# Autodesk Inventor assembly: rapoukAssemblyv2
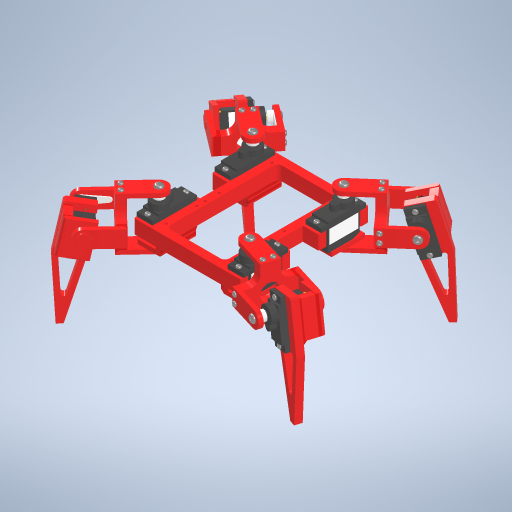
[picture p0: Inventor's stored thumbnail of the model, 512x512]
Saved by Autodesk Inventor 2024 (Build 280153000, 153)
## iProperties
Created: 2024-02-06
Part Number: rapoukAssemblyv2
Document SubType Name: Weldment
Designer: Roman Suk
Weld Material: Welded Aluminum-6061
Author: Roman Suk
## Documents named in this file (9)
- C:\Users\Roman Suk\Documents\Ročníkovka SŠ\CD\Technická dokumentace\rapoukAssemblyv2.iam
- C:\Users\Roman Suk\Documents\Ročníkovka SŠ\CD\Technická dokumentace\rapoukBaseAssemblyv1.iam
- C:\Users\Roman Suk\Documents\Ročníkovka SŠ\CD\Technická dokumentace\сервопривод EMAX ES08MA.ipt
- C:\Users\Roman Suk\Documents\Ročníkovka SŠ\CD\Technická dokumentace\rapoukMiddleLegAssemblyv0.iam
- C:\Users\Roman Suk\Documents\Ročníkovka SŠ\CD\Technická dokumentace\rapoukLegAssemblyv0.iam
- C:\Users\Roman Suk\Documents\Ročníkovka SŠ\CD\Technická dokumentace\rapoukServoLegv0.ipt
- C:\Users\Roman Suk\Documents\Ročníkovka SŠ\CD\Technická dokumentace\rapoukMiddleLeg2v3.ipt
- C:\Users\Roman Suk\Documents\Ročníkovka SŠ\CD\Technická dokumentace\rapoukHexagonScrewM2,5v0.ipt
- C:\Users\Roman Suk\Documents\Ročníkovka SŠ\CD\Technická dokumentace\rapoukHexagonScrewM2v0.ipt
## Components (73 placed, 8 different names)
1. rapoukBaseAssemblyv1:1 [sub-assembly] — Rotational:2, Rotational:4, Rotational:6, Rotational:8, Mate:66, Insert:37, Insert:38, Mate:67, Insert:39, Insert:40, Mate:69, Insert:41, Insert:42, Mate:70, Insert:43, Insert:44
2. сервопривод EMAX ES08MA:1 — Mate:69, Insert:41, Insert:42, Rotational:13, Insert:83, Insert:86
3. сервопривод EMAX ES08MA:2 — Mate:70, Insert:43, Insert:44, Rotational:14, Insert:81, Insert:82
4. сервопривод EMAX ES08MA:3 — Mate:67, Insert:39, Insert:40, Rotational:16, Insert:63, Insert:64
5. сервопривод EMAX ES08MA:4 — Mate:66, Insert:37, Insert:38, Rotational:15, Insert:84, Insert:85
6. rapoukMiddleLegAssemblyv0:3 [sub-assembly] — Insert:21, Insert:22, Insert:23, Insert:24, Rotational:1, Rotational:2
7. rapoukLegAssemblyv0:4 [sub-assembly] — Mate:21, Mate:26, Mate:30, Rotational:1
8. сервопривод EMAX ES08MA:7 — Mate:21, Mate:26, Mate:30, Rotational:9, Insert:71, Insert:72
9. rapoukServoLegv0:4 — Mate:33, Tangent:15, Tangent:16
10. rapoukMiddleLeg2v3:3 — Mate:33, Tangent:15, Tangent:16, Insert:23, Insert:24, Rotational:14, Insert:49, Insert:75, Insert:76
11. rapoukMiddleLeg2v3:5 — Insert:21, Insert:22, Rotational:9, Tangent:29, Tangent:30, Mate:64, Insert:52, Insert:73, Insert:74
12. rapoukMiddleLegAssemblyv0:4 [sub-assembly] — Rotational:4
13. rapoukLegAssemblyv0:5 [sub-assembly]
14. сервопривод EMAX ES08MA:8 — Rotational:10, Insert:69, Insert:70
15. rapoukMiddleLeg2v3:6 — Rotational:13, Mate:73, Tangent:37, Tangent:38, Insert:50, Insert:67, Insert:68
16. rapoukMiddleLeg2v3:7 — Rotational:10, Insert:51, Insert:65, Insert:66
17. rapoukServoLegv0:9
18. rapoukMiddleLegAssemblyv0:5 [sub-assembly] — Rotational:6
19. rapoukLegAssemblyv0:6 [sub-assembly]
20. сервопривод EMAX ES08MA:9 — Rotational:12, Insert:77, Insert:78
21. rapoukMiddleLeg2v3:8 — Rotational:16, Mate:71, Tangent:35, Tangent:36, Insert:48, Insert:59, Insert:60
22. rapoukMiddleLeg2v3:9 — Rotational:12, Tangent:31, Tangent:32, Mate:65, Insert:53, Insert:61, Insert:62
23. rapoukMiddleLegAssemblyv0:6 [sub-assembly] — Rotational:8
24. rapoukLegAssemblyv0:7 [sub-assembly]
25. сервопривод EMAX ES08MA:10 — Rotational:11, Insert:79, Insert:80
26. rapoukMiddleLeg2v3:10 — Rotational:15, Mate:72, Tangent:33, Tangent:34, Insert:47, Insert:55, Insert:56
27. rapoukMiddleLeg2v3:11 — Rotational:11, Insert:54, Insert:57, Insert:58
28. rapoukServoLegv0:11
29. rapoukServoLegv0:12 — Tangent:29, Tangent:30, Mate:64
30. rapoukServoLegv0:13 — Tangent:31, Tangent:32, Mate:65
31. rapoukServoLegv0:14 — Mate:71, Tangent:35, Tangent:36
32. rapoukServoLegv0:15 — Mate:72, Tangent:33, Tangent:34
33. rapoukServoLegv0:17 — Mate:73, Tangent:37, Tangent:38
34. rapoukHexagonScrewM2,5v0:1 — Insert:50
35. rapoukHexagonScrewM2,5v0:2 — Insert:49
36. rapoukHexagonScrewM2,5v0:3 — Insert:48
37. rapoukHexagonScrewM2,5v0:4 — Insert:47
38. rapoukHexagonScrewM2,5v0:5 — Insert:54
39. rapoukHexagonScrewM2,5v0:6 — Insert:53
40. rapoukHexagonScrewM2,5v0:7 — Insert:52
41. rapoukHexagonScrewM2,5v0:8 — Insert:51
42. rapoukHexagonScrewM2v0:1 — Insert:58
43. rapoukHexagonScrewM2v0:2 — Insert:57
44. rapoukHexagonScrewM2v0:3 — Insert:56
45. rapoukHexagonScrewM2v0:4 — Insert:55
46. rapoukHexagonScrewM2v0:5 — Insert:62
47. rapoukHexagonScrewM2v0:6 — Insert:61
48. rapoukHexagonScrewM2v0:7 — Insert:60
49. rapoukHexagonScrewM2v0:8 — Insert:59
50. rapoukHexagonScrewM2v0:9 — Insert:64
51. rapoukHexagonScrewM2v0:10 — Insert:63
52. rapoukHexagonScrewM2v0:11 — Insert:69
53. rapoukHexagonScrewM2v0:12 — Insert:65
54. rapoukHexagonScrewM2v0:13 — Insert:66
55. rapoukHexagonScrewM2v0:14 — Insert:67
56. rapoukHexagonScrewM2v0:15 — Insert:70
57. rapoukHexagonScrewM2v0:16 — Insert:68
58. rapoukHexagonScrewM2v0:17 — Insert:71
59. rapoukHexagonScrewM2v0:18 — Insert:72
60. rapoukHexagonScrewM2v0:19 — Insert:74
61. rapoukHexagonScrewM2v0:20 — Insert:75
62. rapoukHexagonScrewM2v0:21 — Insert:76
63. rapoukHexagonScrewM2v0:22 — Insert:73
64. rapoukHexagonScrewM2v0:23 — Insert:77
65. rapoukHexagonScrewM2v0:24 — Insert:78
66. rapoukHexagonScrewM2v0:25 — Insert:80
67. rapoukHexagonScrewM2v0:26 — Insert:79
68. rapoukHexagonScrewM2v0:27 — Insert:84
69. rapoukHexagonScrewM2v0:28 — Insert:83
70. rapoukHexagonScrewM2v0:29 — Insert:85
71. rapoukHexagonScrewM2v0:30 — Insert:86
72. rapoukHexagonScrewM2v0:31 — Insert:82
73. rapoukHexagonScrewM2v0:32 — Insert:81
## Relationships (120: Insert 64, Mate 24, Tangent 16, RevoluteJoint 16)
- Mate:21: rapoukLegAssemblyv0:4 ↔ сервопривод EMAX ES08MA:7
- Mate:26: rapoukLegAssemblyv0:4 ↔ сервопривод EMAX ES08MA:7
- Mate:30: rapoukLegAssemblyv0:4 ↔ сервопривод EMAX ES08MA:7
- Mate:33: rapoukServoLegv0:4 ↔ rapoukMiddleLeg2v3:3
- Tangent:15: rapoukServoLegv0:4 ↔ rapoukMiddleLeg2v3:3
- Tangent:16: rapoukServoLegv0:4 ↔ rapoukMiddleLeg2v3:3
- Insert:21: rapoukMiddleLegAssemblyv0:3 ↔ rapoukMiddleLeg2v3:5
- Insert:22: rapoukMiddleLegAssemblyv0:3 ↔ rapoukMiddleLeg2v3:5
- Insert:23: rapoukMiddleLegAssemblyv0:3 ↔ rapoukMiddleLeg2v3:3
- Insert:24: rapoukMiddleLegAssemblyv0:3 ↔ rapoukMiddleLeg2v3:3
- Rotational:1 [RevoluteJoint]: rapoukMiddleLegAssemblyv0:3 ↔ rapoukLegAssemblyv0:4
- Rotational:2 [RevoluteJoint] (0.5 mm): rapoukBaseAssemblyv1:1 ↔ rapoukMiddleLegAssemblyv0:3
- [Mate]: rapoukLegAssemblyv0:5 ↔ сервопривод EMAX ES08MA:8
- [Mate]: rapoukLegAssemblyv0:5 ↔ сервопривод EMAX ES08MA:8
- [Mate]: rapoukLegAssemblyv0:5 ↔ сервопривод EMAX ES08MA:8
- [Insert]: rapoukMiddleLegAssemblyv0:4 ↔ rapoukMiddleLeg2v3:7
- [Insert]: rapoukMiddleLegAssemblyv0:4 ↔ rapoukMiddleLeg2v3:7
- [Mate]: rapoukMiddleLeg2v3:7 ↔ rapoukServoLegv0:9
- [Tangent]: rapoukMiddleLeg2v3:7 ↔ rapoukServoLegv0:9
- [Tangent]: rapoukMiddleLeg2v3:7 ↔ rapoukServoLegv0:9
- [Insert]: rapoukMiddleLegAssemblyv0:4 ↔ rapoukMiddleLeg2v3:6
- [Insert]: rapoukMiddleLegAssemblyv0:4 ↔ rapoukMiddleLeg2v3:6
- [RevoluteJoint]: rapoukMiddleLegAssemblyv0:4 ↔ rapoukLegAssemblyv0:5
- Rotational:4 [RevoluteJoint] (-0.5 mm): rapoukBaseAssemblyv1:1 ↔ rapoukMiddleLegAssemblyv0:4
- [Mate]: rapoukLegAssemblyv0:6 ↔ сервопривод EMAX ES08MA:9
- [Mate]: rapoukLegAssemblyv0:6 ↔ сервопривод EMAX ES08MA:9
- [Mate]: rapoukLegAssemblyv0:6 ↔ сервопривод EMAX ES08MA:9
- [Insert]: rapoukMiddleLegAssemblyv0:5 ↔ rapoukMiddleLeg2v3:9
- [Insert]: rapoukMiddleLegAssemblyv0:5 ↔ rapoukMiddleLeg2v3:9
- [Insert]: rapoukMiddleLegAssemblyv0:5 ↔ rapoukMiddleLeg2v3:8
- [Insert]: rapoukMiddleLegAssemblyv0:5 ↔ rapoukMiddleLeg2v3:8
- [RevoluteJoint]: rapoukMiddleLegAssemblyv0:5 ↔ rapoukLegAssemblyv0:6
- Rotational:6 [RevoluteJoint] (-0.5 mm): rapoukBaseAssemblyv1:1 ↔ rapoukMiddleLegAssemblyv0:5
- [Mate]: rapoukLegAssemblyv0:7 ↔ сервопривод EMAX ES08MA:10
- [Mate]: rapoukLegAssemblyv0:7 ↔ сервопривод EMAX ES08MA:10
- [Mate]: rapoukLegAssemblyv0:7 ↔ сервопривод EMAX ES08MA:10
- [Insert]: rapoukMiddleLegAssemblyv0:6 ↔ rapoukMiddleLeg2v3:11
- [Insert]: rapoukMiddleLegAssemblyv0:6 ↔ rapoukMiddleLeg2v3:11
- [Mate]: rapoukMiddleLeg2v3:11 ↔ rapoukServoLegv0:11
- [Tangent]: rapoukMiddleLeg2v3:11 ↔ rapoukServoLegv0:11
- [Tangent]: rapoukMiddleLeg2v3:11 ↔ rapoukServoLegv0:11
- [Insert]: rapoukMiddleLegAssemblyv0:6 ↔ rapoukMiddleLeg2v3:10
- [Insert]: rapoukMiddleLegAssemblyv0:6 ↔ rapoukMiddleLeg2v3:10
- [RevoluteJoint]: rapoukMiddleLegAssemblyv0:6 ↔ rapoukLegAssemblyv0:7
- Rotational:8 [RevoluteJoint] (0.5 mm): rapoukBaseAssemblyv1:1 ↔ rapoukMiddleLegAssemblyv0:6
- Rotational:9 [RevoluteJoint] (-4.3 mm): сервопривод EMAX ES08MA:7 ↔ rapoukMiddleLeg2v3:5
- Tangent:29: rapoukMiddleLeg2v3:5 ↔ rapoukServoLegv0:12
- Tangent:30: rapoukMiddleLeg2v3:5 ↔ rapoukServoLegv0:12
- Mate:64: rapoukMiddleLeg2v3:5 ↔ rapoukServoLegv0:12
- Rotational:10 [RevoluteJoint] (4.3 mm): сервопривод EMAX ES08MA:8 ↔ rapoukMiddleLeg2v3:7
- Rotational:11 [RevoluteJoint] (-4.3 mm): сервопривод EMAX ES08MA:10 ↔ rapoukMiddleLeg2v3:11
- Rotational:12 [RevoluteJoint] (-4.3 mm): сервопривод EMAX ES08MA:9 ↔ rapoukMiddleLeg2v3:9
- Tangent:31: rapoukMiddleLeg2v3:9 ↔ rapoukServoLegv0:13
- Tangent:32: rapoukMiddleLeg2v3:9 ↔ rapoukServoLegv0:13
- Mate:65: rapoukMiddleLeg2v3:9 ↔ rapoukServoLegv0:13
- Mate:66: rapoukBaseAssemblyv1:1 ↔ сервопривод EMAX ES08MA:4
- Insert:37: rapoukBaseAssemblyv1:1 ↔ сервопривод EMAX ES08MA:4
- Insert:38: rapoukBaseAssemblyv1:1 ↔ сервопривод EMAX ES08MA:4
- Mate:67: rapoukBaseAssemblyv1:1 ↔ сервопривод EMAX ES08MA:3
- Insert:39: rapoukBaseAssemblyv1:1 ↔ сервопривод EMAX ES08MA:3
- Insert:40: rapoukBaseAssemblyv1:1 ↔ сервопривод EMAX ES08MA:3
- Mate:69: rapoukBaseAssemblyv1:1 ↔ сервопривод EMAX ES08MA:1
- Insert:41: rapoukBaseAssemblyv1:1 ↔ сервопривод EMAX ES08MA:1
- Insert:42: rapoukBaseAssemblyv1:1 ↔ сервопривод EMAX ES08MA:1
- Mate:70: rapoukBaseAssemblyv1:1 ↔ сервопривод EMAX ES08MA:2
- Insert:43: rapoukBaseAssemblyv1:1 ↔ сервопривод EMAX ES08MA:2
- Insert:44: rapoukBaseAssemblyv1:1 ↔ сервопривод EMAX ES08MA:2
- Rotational:13 [RevoluteJoint] (4.3 mm): сервопривод EMAX ES08MA:1 ↔ rapoukMiddleLeg2v3:6
- Rotational:14 [RevoluteJoint] (4.3 mm): сервопривод EMAX ES08MA:2 ↔ rapoukMiddleLeg2v3:3
- Rotational:15 [RevoluteJoint] (4.3 mm): сервопривод EMAX ES08MA:4 ↔ rapoukMiddleLeg2v3:10
- Rotational:16 [RevoluteJoint] (4.3 mm): сервопривод EMAX ES08MA:3 ↔ rapoukMiddleLeg2v3:8
- Mate:71: rapoukMiddleLeg2v3:8 ↔ rapoukServoLegv0:14
- Mate:72: rapoukMiddleLeg2v3:10 ↔ rapoukServoLegv0:15
- Tangent:33: rapoukMiddleLeg2v3:10 ↔ rapoukServoLegv0:15
- Tangent:34: rapoukMiddleLeg2v3:10 ↔ rapoukServoLegv0:15
- Tangent:35: rapoukMiddleLeg2v3:8 ↔ rapoukServoLegv0:14
- Tangent:36: rapoukMiddleLeg2v3:8 ↔ rapoukServoLegv0:14
- Mate:73: rapoukMiddleLeg2v3:6 ↔ rapoukServoLegv0:17
- Tangent:37: rapoukMiddleLeg2v3:6 ↔ rapoukServoLegv0:17
- Tangent:38: rapoukMiddleLeg2v3:6 ↔ rapoukServoLegv0:17
- Insert:47: rapoukMiddleLeg2v3:10 ↔ rapoukHexagonScrewM2,5v0:4
- Insert:48: rapoukMiddleLeg2v3:8 ↔ rapoukHexagonScrewM2,5v0:3
- Insert:49: rapoukMiddleLeg2v3:3 ↔ rapoukHexagonScrewM2,5v0:2
- Insert:50: rapoukMiddleLeg2v3:6 ↔ rapoukHexagonScrewM2,5v0:1
- Insert:51: rapoukMiddleLeg2v3:7 ↔ rapoukHexagonScrewM2,5v0:8
- Insert:52: rapoukMiddleLeg2v3:5 ↔ rapoukHexagonScrewM2,5v0:7
- Insert:53: rapoukMiddleLeg2v3:9 ↔ rapoukHexagonScrewM2,5v0:6
- Insert:54: rapoukMiddleLeg2v3:11 ↔ rapoukHexagonScrewM2,5v0:5
- Insert:55: rapoukMiddleLeg2v3:10 ↔ rapoukHexagonScrewM2v0:4
- Insert:56: rapoukMiddleLeg2v3:10 ↔ rapoukHexagonScrewM2v0:3
- Insert:57: rapoukMiddleLeg2v3:11 ↔ rapoukHexagonScrewM2v0:2
- Insert:58: rapoukMiddleLeg2v3:11 ↔ rapoukHexagonScrewM2v0:1
- Insert:59: rapoukMiddleLeg2v3:8 ↔ rapoukHexagonScrewM2v0:8
- Insert:60: rapoukMiddleLeg2v3:8 ↔ rapoukHexagonScrewM2v0:7
- Insert:61: rapoukMiddleLeg2v3:9 ↔ rapoukHexagonScrewM2v0:6
- Insert:62: rapoukMiddleLeg2v3:9 ↔ rapoukHexagonScrewM2v0:5
- Insert:63: сервопривод EMAX ES08MA:3 ↔ rapoukHexagonScrewM2v0:10
- Insert:64: сервопривод EMAX ES08MA:3 ↔ rapoukHexagonScrewM2v0:9
- Insert:65: rapoukMiddleLeg2v3:7 ↔ rapoukHexagonScrewM2v0:12
- Insert:66: rapoukMiddleLeg2v3:7 ↔ rapoukHexagonScrewM2v0:13
- Insert:67: rapoukMiddleLeg2v3:6 ↔ rapoukHexagonScrewM2v0:14
- Insert:68: rapoukMiddleLeg2v3:6 ↔ rapoukHexagonScrewM2v0:16
- Insert:69: сервопривод EMAX ES08MA:8 ↔ rapoukHexagonScrewM2v0:11
- Insert:70: сервопривод EMAX ES08MA:8 ↔ rapoukHexagonScrewM2v0:15
- Insert:71: сервопривод EMAX ES08MA:7 ↔ rapoukHexagonScrewM2v0:17
- Insert:72: сервопривод EMAX ES08MA:7 ↔ rapoukHexagonScrewM2v0:18
- Insert:73: rapoukMiddleLeg2v3:5 ↔ rapoukHexagonScrewM2v0:22
- Insert:74: rapoukMiddleLeg2v3:5 ↔ rapoukHexagonScrewM2v0:19
- Insert:75: rapoukMiddleLeg2v3:3 ↔ rapoukHexagonScrewM2v0:20
- Insert:76: rapoukMiddleLeg2v3:3 ↔ rapoukHexagonScrewM2v0:21
- Insert:77: сервопривод EMAX ES08MA:9 ↔ rapoukHexagonScrewM2v0:23
- Insert:78: сервопривод EMAX ES08MA:9 ↔ rapoukHexagonScrewM2v0:24
- Insert:79: сервопривод EMAX ES08MA:10 ↔ rapoukHexagonScrewM2v0:26
- Insert:80: сервопривод EMAX ES08MA:10 ↔ rapoukHexagonScrewM2v0:25
- Insert:81: сервопривод EMAX ES08MA:2 ↔ rapoukHexagonScrewM2v0:32
- Insert:82: сервопривод EMAX ES08MA:2 ↔ rapoukHexagonScrewM2v0:31
- Insert:83: сервопривод EMAX ES08MA:1 ↔ rapoukHexagonScrewM2v0:28
- Insert:84: сервопривод EMAX ES08MA:4 ↔ rapoukHexagonScrewM2v0:27
- Insert:85: сервопривод EMAX ES08MA:4 ↔ rapoukHexagonScrewM2v0:29
- Insert:86: сервопривод EMAX ES08MA:1 ↔ rapoukHexagonScrewM2v0:30
## Named parameters: d151_d135 = 0 mm, d152_d136 = 0 mm, d153_d139 = 0 mm, d154_d140 = 0 mm, d155_d147 = 0 mm, d156_d148 = 100.953704 deg, d157_d60 = 0 mm, d158_d64 = 0 mm, d159_d131 = 0 mm, d160_d132 = 0 mm, d161_d134 = 0 mm, d162_d55 = 0 mm, d167_d139 = 0 mm, d168_d140 = 0 mm, d169_d147 = 0 mm, d170_d148 = 105.713773 deg, d171_d60 = 0 mm, d172_d64 = 0 mm, d173_d131 = 0 mm, d174_d132 = 0 mm, d176_d55 = 0 mm, d179_d135 = 0 mm, d180_d136 = 0 mm, d181_d139 = 0 mm, d182_d140 = 0 mm, d183_d147 = 0 mm, d184_d148 = 100.743768 deg, d185_d60 = 0 mm, d186_d64 = 0 mm, d187_d131 = 0 mm, d188_d132 = 0 mm, d189_d134 = 0 mm, d190_d55 = 0 mm
